# Autodesk Inventor assembly: threadTest
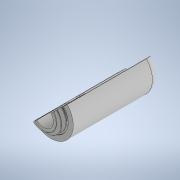
[picture p0: Inventor's stored thumbnail of the model, 180x180]
Saved by Autodesk Inventor 2022 (Build 260153000, 153)
## iProperties
Created: 2021-10-07
Part Number: threadTest
Document SubType Name: Assembly
Designer: tecware
Author: tecware
## Documents named in this file (3)
- C:\Users\tecware\Documents\Inventor\activeMarker\wand\threadTest\threadTest.iam
- C:\Users\tecware\Documents\Inventor\activeMarker\wand\threadTest\thread-m.ipt
- C:\Users\tecware\Documents\Inventor\activeMarker\wand\threadTest\thread-f.ipt
## Components (2 placed, 2 different names)
1. thread-m:1 — Mate:1
2. thread-f:1 — Mate:1
## Relationships (1: Mate 1)
- Mate:1: thread-m:1 ↔ thread-f:1
